# Autodesk Inventor assembly: ASY BSH 610 reagent dosator
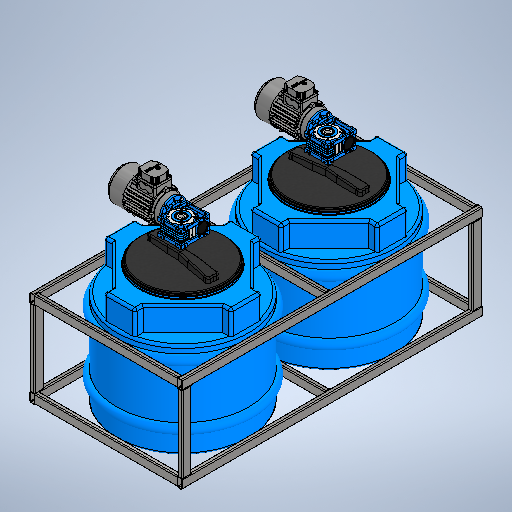
[picture p0: Inventor's stored thumbnail of the model, 512x512]
Saved by Autodesk Inventor 2025 (Build 290162010, 162A)
## iProperties
Created: 2024-09-22
Part Number: ASY BSH 610 reagent dosator
Document SubType Name: Assembly
Designer: admin
Author: admin
## Documents named in this file (5)
- C:\Users\admin\YandexDisk-badmisterfox\домашниий пк\Inventor\BSH_Beshkino_bio_tank\ASY BSH 610 reagent dosator.iam
- C:\Users\admin\YandexDisk-badmisterfox\домашниий пк\Inventor\BSH_Beshkino_bio_tank\BSH 12 reagent tank.ipt
- C:\Users\admin\YandexDisk-badmisterfox\домашниий пк\Inventor\BSH_Beshkino_bio_tank\ASY BSH tank frame.iam
- C:\Users\admin\YandexDisk-badmisterfox\домашниий пк\Inventor\BSH_Beshkino_bio_tank\1.1 крышка.ipt
- C:\Users\admin\YandexDisk-badmisterfox\домашниий пк\Inventor\BSH_Beshkino_bio_tank\3d party\motor-reductor NMRV040\motor-reductor NMRV040.iam
## Components (7 placed, 4 different names)
1. ASY BSH tank frame:1 [sub-assembly] — Tangent:1, Tangent:2, Mate:5
2. BSH 12 reagent tank:2 — Mate:2, Mate:3, Tangent:2, Rigid:1
3. BSH 12 reagent tank:1 — Rigid:2, Mate:1, Mate:4, Tangent:1
4. 1.1 крышка:1 — Rigid:2
5. 1.1 крышка:2 — Rigid:1
6. motor-reductor NMRV040:1 [sub-assembly] — Flush:1, Flush:3, Mate:5
7. motor-reductor NMRV040:2 [sub-assembly] — Flush:2, Flush:3
## Relationships (12: Mate 5, Flush 3, WeldJoint 2, Tangent 2)
- Rigid:2 [WeldJoint]: BSH 12 reagent tank:1 ↔ 1.1 крышка:1
- Mate:1: BSH 12 reagent tank:1
- Mate:2: BSH 12 reagent tank:2
- Mate:3: BSH 12 reagent tank:2
- Mate:4: BSH 12 reagent tank:1
- Tangent:1: ASY BSH tank frame:1 ↔ BSH 12 reagent tank:1
- Tangent:2: ASY BSH tank frame:1 ↔ BSH 12 reagent tank:2
- Rigid:1 [WeldJoint]: BSH 12 reagent tank:2 ↔ 1.1 крышка:2
- Flush:1: motor-reductor NMRV040:1
- Flush:2: motor-reductor NMRV040:2
- Flush:3: motor-reductor NMRV040:1 ↔ motor-reductor NMRV040:2
- Mate:5 (200 mm): ASY BSH tank frame:1 ↔ motor-reductor NMRV040:1
